# Autodesk Inventor assembly: wheelholder1
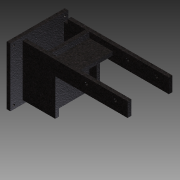
[picture p0: Inventor's stored thumbnail of the model, 180x180]
Saved by Autodesk Inventor 2011 (Build 150239000, 239)
## iProperties
Created: 2011-09-17
Part Number: wheelholder1
Document SubType Name: Assembly
Designer: Matthew
Author: Matthew
## Documents named in this file (6)
- C:\Users\Matthew\Documents\matthew_autocad\prlite\wheel\wheelholder1.iam
- C:\Users\Matthew\Documents\matthew_autocad\prlite\wheel\side 2.ipt
- C:\Users\Matthew\Documents\matthew_autocad\prlite\wheel\side 1.ipt
- C:\Users\Matthew\Documents\matthew_autocad\prlite\wheel\support 1.ipt
- C:\Users\Matthew\Documents\matthew_autocad\prlite\wheel\support 2.ipt
- C:\Users\Matthew\Documents\matthew_autocad\prlite\wheel\wheel top.ipt
## Components (5 placed, 5 different names)
1. side 2:1 — Mate:1, Flush:1, Mate:2, Flush:3, Mate:5, Mate:6
2. side 1:1 — Flush:2, Mate:3, Mate:4, Flush:5
3. support 1:1 — Flush:3, Mate:5, Mate:6, Flush:4, Mate:7
4. support 2:1 — Flush:4, Flush:5, Mate:7
5. wheel top:1 — Mate:1, Flush:1, Mate:2, Flush:2, Mate:3, Mate:4
## Relationships (12: Mate 7, Flush 5)
- Mate:1: side 2:1 ↔ wheel top:1
- Flush:1: side 2:1 ↔ wheel top:1
- Mate:2: side 2:1 ↔ wheel top:1
- Flush:2: side 1:1 ↔ wheel top:1
- Mate:3: side 1:1 ↔ wheel top:1
- Mate:4: side 1:1 ↔ wheel top:1
- Flush:3: side 2:1 ↔ support 1:1
- Mate:5: side 2:1 ↔ support 1:1
- Mate:6: side 2:1 ↔ support 1:1
- Flush:4: support 1:1 ↔ support 2:1
- Flush:5: side 1:1 ↔ support 2:1
- Mate:7: support 1:1 ↔ support 2:1
